# Autodesk Inventor assembly: MECHANICAL ARM
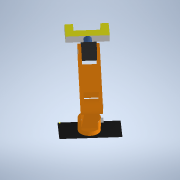
[picture p0: Inventor's stored thumbnail of the model, 180x180]
Saved by Autodesk Inventor 2021 (Build 250183000, 183)
## iProperties
Created: 2021-07-24
Part Number: MECHANICAL ARM
Document SubType Name: Assembly
Designer: aksha
Author: aksha
## Documents named in this file (7)
- C:\akshu\Autodesk\BHUVAN MECHANICAL-ARM\MECHANICAL ARM (1).iam
- C:\akshu\Autodesk\BHUVAN MECHANICAL-ARM\Part1.ipt
- C:\akshu\Autodesk\BHUVAN MECHANICAL-ARM\FIRST ARM.ipt
- C:\akshu\Autodesk\BHUVAN MECHANICAL-ARM\PIN-1.ipt
- C:\akshu\Autodesk\BHUVAN MECHANICAL-ARM\SECOND ARM.ipt
- C:\akshu\Autodesk\BHUVAN MECHANICAL-ARM\HOLDER.ipt
- C:\akshu\Autodesk\BHUVAN MECHANICAL-ARM\PIN-2.ipt
## Components (7 placed, 6 different names)
1. Part1:1 — Mate:1
2. FIRST ARM:1 — Mate:1, Mate:2, Mate:3, Mate:6
3. PIN-1:1 — Mate:2
4. SECOND ARM:1 — Mate:3, Mate:4, Mate:7, Angle:1
5. HOLDER:1 — Mate:4, Mate:5, Angle:1
6. PIN-2:1 — Mate:6
7. PIN-2:2 — Mate:5, Mate:7
## Relationships (8: Mate 7, Angle 1)
- Mate:1: Part1:1 ↔ FIRST ARM:1
- Mate:2: FIRST ARM:1 ↔ PIN-1:1
- Mate:3: FIRST ARM:1 ↔ SECOND ARM:1
- Mate:4: SECOND ARM:1 ↔ HOLDER:1
- Mate:5: HOLDER:1 ↔ PIN-2:2
- Mate:6: FIRST ARM:1 ↔ PIN-2:1
- Mate:7: SECOND ARM:1 ↔ PIN-2:2
- Angle:1 (0 deg): SECOND ARM:1 ↔ HOLDER:1
